# Autodesk Inventor assembly: Assembly
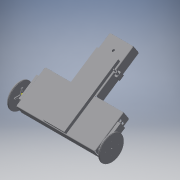
[picture p0: Inventor's stored thumbnail of the model, 180x180]
Saved by Autodesk Inventor 2016 (Build 200138000, 138)
## iProperties
Created: 2016-10-21
Part Number: Assembly
Document SubType Name: Assembly
Designer: sheehm
Author: sheehm
## Documents named in this file (11)
- E:\Line Tracking Robot\Assembly.iam
- E:\Line Tracking Robot\Frame.ipt
- E:\Line Tracking Robot\Serial Motor.ipt
- E:\Line Tracking Robot\Servo Horn.ipt
- E:\Line Tracking Robot\Wheel.ipt
- E:\Line Tracking Robot\Battery Pack.ipt
- E:\Line Tracking Robot\Bread Board.ipt
- E:\Line Tracking Robot\Caster.ipt
- E:\Line Tracking Robot\Marble.ipt
- E:\Line Tracking Robot\Switch.ipt
- E:\Line Tracking Robot\O-Ring.ipt
## Components (14 placed, 10 different names)
1. Frame:1 — Rigid:1, Rigid:2, Rigid:3, Rigid:7, Rigid:8
2. Serial Motor:1 — Rigid:1, Rotational:2
3. Serial Motor:2 — Rigid:2, Rotational:1
4. Servo Horn:1 — Rotational:1, Rotational:4
5. Servo Horn:2 — Rotational:2, Rotational:5
6. Caster:1 — Rigid:3, Ball:1
7. Marble:1 — Ball:1
8. Battery Pack:1 — Rigid:8
9. Switch:1 — Rigid:7
10. Bread Board:1
11. Wheel:2 — Rotational:4, Rigid:10
12. O-Ring:6 — Rigid:10
13. Wheel:3 — Rotational:5, Rigid:11
14. O-Ring:7 — Rigid:11
## Relationships (16: WeldJoint 7, RevoluteJoint 4, Flush 4, BallJoint 1)
- Rigid:1 [WeldJoint]: Frame:1 ↔ Serial Motor:1
- Rigid:2 [WeldJoint]: Frame:1 ↔ Serial Motor:2
- Rotational:1 [RevoluteJoint]: Serial Motor:2 ↔ Servo Horn:1
- Rotational:2 [RevoluteJoint]: Serial Motor:1 ↔ Servo Horn:2
- Flush:1 (-27.686 mm)
- Flush:2 (-43.1038 mm)
- Flush:3 (-42.1615 mm)
- Flush:4 (-36.195 mm)
- Rigid:3 [WeldJoint]: Frame:1 ↔ Caster:1
- Ball:1: Caster:1 ↔ Marble:1
- Rigid:7 [WeldJoint]: Frame:1 ↔ Switch:1
- Rigid:8 [WeldJoint]: Frame:1 ↔ Battery Pack:1
- Rotational:4 [RevoluteJoint]: Servo Horn:1 ↔ Wheel:2
- Rigid:10 [WeldJoint]: Wheel:2 ↔ O-Ring:6
- Rotational:5 [RevoluteJoint]: Servo Horn:2 ↔ Wheel:3
- Rigid:11 [WeldJoint]: Wheel:3 ↔ O-Ring:7
